# Autodesk Inventor assembly: LowerFrontLink
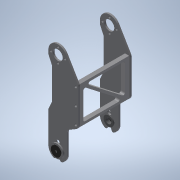
[picture p0: Inventor's stored thumbnail of the model, 180x180]
Saved by Autodesk Inventor 2020.4 (Build 244396000, 396)
## iProperties
Created: 2016-08-23
Part Number: LowerFrontLink
Material: 一般
Document SubType Name: Assembly
Designer: hiro
Mass: 33.5175 g
Surface Area: 182.778 cm^2
Volume: 15.549 cm^3
Density: 2.15561 g/cm^3
Author: hiro
## Documents named in this file (6)
- C:\Users\Masato\Documents\Inventor\CIT Brains_Inventor\名称変更\OpenPlatform_ver3_0\LowerBody\リンク\LowerFrontLink.iam
- C:\Users\Masato\Documents\Inventor\CIT Brains_Inventor\名称変更\OpenPlatform_ver3_0\LowerBody\リンク\Link_front_diagonal.ipt
- C:\Users\Masato\Documents\Inventor\CIT Brains_Inventor\名称変更\OpenPlatform_ver3_0\LowerBody\リンク\Link_front_side_frame.ipt
- C:\Users\Masato\Documents\Inventor\CIT Brains_Inventor\名称変更\OpenPlatform_ver3_0\Ready_Made\LFW-0815.ipt
- C:\Users\Masato\Documents\Inventor\CIT Brains_Inventor\名称変更\OpenPlatform_ver3_0\Ready_Made\UUW-0312-10BH.ipt
- C:\Users\Masato\Documents\Inventor\CIT Brains_Inventor\名称変更\OpenPlatform_ver3_0\Ready_Made\80F-0603.ipt
## Components (9 placed, 5 different names)
1. Link_front_side_frame:1 — 挿入:7, 挿入:8, 挿入:9, 挿入:13, 挿入:17
2. Link_front_side_frame:2 — 挿入:10, 挿入:11, 挿入:12, 挿入:14, 挿入:18
3. Link_front_diagonal:1 — 挿入:7, 挿入:8, 挿入:9, 挿入:10, 挿入:11, 挿入:12
4. LFW-0815:1 — 挿入:13, 挿入:16
5. LFW-0815:2 — 挿入:14, 挿入:15
6. UUW-0312-10BH:1 — 挿入:16
7. UUW-0312-10BH:2 — 挿入:15
8. 80F-0603:1 — 挿入:17
9. 80F-0603:2 — 挿入:18
## Relationships (12: Insert 12)
- 挿入:7 [Insert]: Link_front_side_frame:1 ↔ Link_front_diagonal:1
- 挿入:8 [Insert]: Link_front_side_frame:1 ↔ Link_front_diagonal:1
- 挿入:9 [Insert]: Link_front_side_frame:1 ↔ Link_front_diagonal:1
- 挿入:10 [Insert]: Link_front_side_frame:2 ↔ Link_front_diagonal:1
- 挿入:11 [Insert]: Link_front_side_frame:2 ↔ Link_front_diagonal:1
- 挿入:12 [Insert]: Link_front_side_frame:2 ↔ Link_front_diagonal:1
- 挿入:13 [Insert]: Link_front_side_frame:1 ↔ LFW-0815:1
- 挿入:14 [Insert]: Link_front_side_frame:2 ↔ LFW-0815:2
- 挿入:15 [Insert]: LFW-0815:2 ↔ UUW-0312-10BH:2
- 挿入:16 [Insert]: LFW-0815:1 ↔ UUW-0312-10BH:1
- 挿入:17 [Insert]: Link_front_side_frame:1 ↔ 80F-0603:1
- 挿入:18 [Insert]: Link_front_side_frame:2 ↔ 80F-0603:2
